# Autodesk Inventor assembly: Ensamblaje1
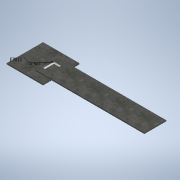
[picture p0: Inventor's stored thumbnail of the model, 180x180]
Saved by Autodesk Inventor 2020.5 (Build 245400000, 400)
## iProperties
Created: 2023-01-30
Part Number: Ensamblaje1
Document SubType Name: Conjunto soldado
Designer: André Aguirre Apolo
Weld Material: Aluminio 6061, soldado
Author: André Aguirre Apolo
## Documents named in this file (4)
- C:\Users\André Aguirre Apolo\Desktop\ESPOL\PAO2, 2022\Diseño y simulacion de maquinas\Teorico\Tareasoldadura\Ensamblaje1.iam
- C:\Users\André Aguirre Apolo\Desktop\ESPOL\PAO2, 2022\Diseño y simulacion de maquinas\Teorico\Tareasoldadura\Pieza1.ipt
- C:\Users\André Aguirre Apolo\Desktop\ESPOL\PAO2, 2022\Diseño y simulacion de maquinas\Teorico\Tareasoldadura\Pieza2.ipt
- C:\Users\André Aguirre Apolo\Desktop\ESPOL\PAO2, 2022\Diseño y simulacion de maquinas\Teorico\Tareasoldadura\Ensamblaje1\Design Accelerator\Soldadura de empalme (carga en plano de conexión)1.iam
## Components (3 placed, 3 different names)
1. Pieza1:1 — Coincidencia:1
2. Pieza2:1 — Coincidencia:1
3. Soldadura de empalme (carga en plano de conexión):1 [sub-assembly]
## Relationships (1: Mate 1)
- Coincidencia:1 [Mate]: Pieza1:1 ↔ Pieza2:1
